# Autodesk Inventor assembly: asmTemp
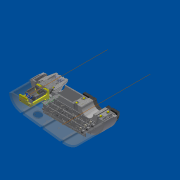
[picture p0: Inventor's stored thumbnail of the model, 180x180]
Saved by Autodesk Inventor 2018 (Build 220112000, 112)
## iProperties
Created: 2019-11-13
Part Number: asmTemp
Document SubType Name: Assembly
Designer: Bunny320
Author: Bunny320
## Documents named in this file (22)
- C:\Users\Bunny320\Desktop\sechs\4-CAD\10-J1.iam
- C:\Users\Bunny320\Desktop\sechs\4-CAD\generated\J1_belt.iam
- C:\Users\Bunny320\Desktop\sechs\4-CAD\standardParts\61814-2RS1\61814-2RS1.iam
- C:\Users\Bunny320\Desktop\sechs\4-CAD\AS5047.ipt
- C:\Users\Bunny320\Desktop\sechs\4-CAD\standardParts\SUNNYSKY-X6215S-kv170\X6215S.ipt
- C:\Users\Bunny320\Desktop\sechs\4-CAD\104-motor-case-new.ipt
- C:\Users\Bunny320\Desktop\sechs\4-CAD\102-top-motor-adapt-big-motor.ipt
- C:\Users\Bunny320\Desktop\sechs\4-CAD\105-flange adapter.ipt
- C:\Users\Bunny320\Documents\Inventor\Content Center Files\R2018\en-US\ISO 10642(2)\ISO 10642  - M3  x  20.ipt
- C:\Users\Bunny320\Documents\Inventor\Content Center Files\R2018\en-US\ISO 4762(1)\DIN EN ISO 4762 - M2 x 6.ipt
- C:\Users\Bunny320\Documents\Inventor\Content Center Files\R2018\en-US\DIN EN ISO 4032\DIN EN ISO 4032 - M2.ipt
- C:\Users\Bunny320\Documents\Inventor\Content Center Files\R2018\en-US\ISO 10642(2)\ISO 10642  - M4  x  16.ipt
- C:\Users\Bunny320\Documents\Inventor\Content Center Files\R2018\en-US\ISO 4762(1)\DIN EN ISO 4762 - M3 x 10.ipt
- C:\Users\Bunny320\Desktop\sechs\4-CAD\standardParts\Pololu mounting hub\pololu-universal-aluminum-mounting-hub-for-6mm-shaft-m3-holes.ipt
- C:\Users\Bunny320\Desktop\sechs\4-CAD\standardParts\61807-2RS1\61807-2RS1.iam
- C:\Users\Bunny320\Desktop\sechs\4-CAD\generated\J1_belt\Design Accelerator\Synchronous Pulley11.ipt
- C:\Users\Bunny320\Desktop\sechs\4-CAD\standardParts\Odrive\PCBasembly_simp.ipt
- C:\Users\Bunny320\Desktop\sechs\4-CAD\motor unit 2820 (J1).iam
- C:\Users\Bunny320\Desktop\sechs\4-CAD\106-pulley adapter.ipt
- C:\Users\Bunny320\Desktop\sechs\4-CAD\112-base middle.ipt
- C:\Users\Bunny320\Desktop\sechs\4-CAD\113-base bottom.ipt
- C:\Users\Bunny320\Desktop\sechs\4-CAD\114-base top.ipt
## Components (47 placed, 21 different names)
1. 112-base middle:1 — Mate:5, Mate:28, Mate:102, Mate:107, Mate:108, Mate:109, Mate:111, Mate:112, Mate:113
2. J1_belt:1 [sub-assembly] — Mate:1, Mate:2, Mate:3, Mate:6, Mate:7, Mate:8, Mate:20, Mate:26, Mate:27, Mate:30, Mate:32, Mate:33, Mate:34, Mate:35, Mate:101, Mate:105, Mate:106
3. 61814-2RS1:1 [sub-assembly] — Mate:2, Mate:8, Mate:110
4. 61814-2RS1:2 [sub-assembly] — Mate:3, Mate:5, Mate:7
5. AS5047:1 — Mate:21, Mate:22, Mate:23, Mate:37, Mate:39, Mate:41, Mate:43
6. X6215S:1 — Mate:24, Mate:25, Mate:26
7. 104-motor-case-new:1 — Mate:20, Mate:21, Mate:22, Mate:23, Mate:24, Mate:25, Mate:36, Mate:38, Mate:40, Mate:42, Mate:45, Mate:47, Mate:49, Mate:51, Mate:52
8. 102-top-motor-adapt-big-motor:1 — Mate:27, Mate:28, Mate:29, Mate:53, Mate:54, Mate:55, Mate:56, Mate:57, Mate:58, Mate:59, Mate:60, Mate:61, Mate:62, Mate:63, Mate:64, Mate:66, Mate:68, Mate:70, Mate:72, Mate:74, Mate:76, Mate:78
9. 105-flange adapter:1 — Mate:30, Mate:105, Mate:106
10. DIN EN ISO 10642 M3  x  20:1 — Mate:32
11. DIN EN ISO 10642 M3  x  20:2 — Mate:33
12. DIN EN ISO 10642 M3  x  20:3 — Mate:34
13. DIN EN ISO 10642 M3  x  20:4 — Mate:35
14. DIN EN ISO 4762 M2 x 6:1 — Mate:36, Mate:37, Mate:50
15. DIN EN ISO 4762 M2 x 6:2 — Mate:38, Mate:39, Mate:46
16. DIN EN ISO 4762 M2 x 6:3 — Mate:40, Mate:41, Mate:44
17. DIN EN ISO 4762 M2 x 6:4 — Mate:42, Mate:43, Mate:48
18. DIN EN ISO 4032 M2:1 — Mate:44, Mate:45
19. DIN EN ISO 4032 M2:2 — Mate:46, Mate:47
20. DIN EN ISO 4032 M2:3 — Mate:48, Mate:49
21. DIN EN ISO 4032 M2:4 — Mate:50, Mate:51
22. DIN EN ISO 4762 M3 x 10:1 — Mate:53, Mate:54
23. DIN EN ISO 4762 M3 x 10:2 — Mate:55, Mate:56
24. DIN EN ISO 4762 M3 x 10:3 — Mate:57, Mate:58
25. DIN EN ISO 4762 M3 x 10:4 — Mate:59, Mate:60
26. DIN EN ISO 4762 M3 x 10:5 — Mate:61, Mate:62
27. DIN EN ISO 4762 M3 x 10:6 — Mate:63, Mate:64
28. DIN EN ISO 4762 M3 x 10:7 — Mate:66
29. DIN EN ISO 4762 M3 x 10:8 — Mate:68
30. DIN EN ISO 4762 M3 x 10:9 — Mate:70
31. DIN EN ISO 4762 M3 x 10:10 — Mate:72
32. DIN EN ISO 4762 M3 x 10:11 — Mate:74
33. DIN EN ISO 4762 M3 x 10:12 — Mate:76
34. DIN EN ISO 4762 M3 x 10:13 — Mate:78
35. motor unit 2820 (J1):1 [sub-assembly] — Flush:4, Mate:92, Mate:100, Mate:101, Mate:102
36. pololu-universal-aluminum-mounting-hub-for-6mm-shaft-m3-holes:1 — Flush:4, Mate:92, Mate:97
37. 61807-2RS1:1 [sub-assembly] — Mate:98, Mate:99, Mate:100, Mate:103, Mate:104
38. Synchronous Pulley1:1 — Mate:97, Mate:98, Mate:99
39. PCBasembly_simp:1 — Mate:112, Mate:113
40. 106-pulley adapter:1 — Mate:103, Mate:104
41. 113-base bottom:1 — Mate:107, Mate:108, Mate:109
42. 114-base top:1 — Mate:110, Mate:111
43. PCBasembly_simp:2
44. PCBasembly_simp:3
45. DIN EN ISO 10642 M4  x  16:1 — Mate:52
46. DIN EN ISO 10642 M4  x  16:2
47. DIN EN ISO 10642 M4  x  16:3
## Component patterns: (4 elements, first: DIN EN ISO 10642 M4  x  16:1)
## Relationships (80: Mate 76, Flush 4)
- [Flush]: 112-base middle:1
- [Flush]: 112-base middle:1
- [Flush]: 112-base middle:1
- Mate:1: J1_belt:1
- Mate:2: J1_belt:1 ↔ 61814-2RS1:1
- Mate:3: J1_belt:1 ↔ 61814-2RS1:2
- Mate:5: 112-base middle:1 ↔ 61814-2RS1:2
- Mate:6: J1_belt:1
- Mate:7: J1_belt:1 ↔ 61814-2RS1:2
- Mate:8: J1_belt:1 ↔ 61814-2RS1:1
- Mate:20: J1_belt:1 ↔ 104-motor-case-new:1
- Mate:21: AS5047:1 ↔ 104-motor-case-new:1
- Mate:22: AS5047:1 ↔ 104-motor-case-new:1
- Mate:23: AS5047:1 ↔ 104-motor-case-new:1
- Mate:24: X6215S:1 ↔ 104-motor-case-new:1
- Mate:25: X6215S:1 ↔ 104-motor-case-new:1
- Mate:26: J1_belt:1 ↔ X6215S:1
- Mate:27: J1_belt:1 ↔ 102-top-motor-adapt-big-motor:1
- Mate:28: 112-base middle:1 ↔ 102-top-motor-adapt-big-motor:1
- Mate:29: 102-top-motor-adapt-big-motor:1
- Mate:30: J1_belt:1 ↔ 105-flange adapter:1
- Mate:32: J1_belt:1 ↔ DIN EN ISO 10642 M3  x  20:1
- Mate:33: J1_belt:1 ↔ DIN EN ISO 10642 M3  x  20:2
- Mate:34: J1_belt:1 ↔ DIN EN ISO 10642 M3  x  20:3
- Mate:35: J1_belt:1 ↔ DIN EN ISO 10642 M3  x  20:4
- Mate:36: 104-motor-case-new:1 ↔ DIN EN ISO 4762 M2 x 6:1
- Mate:37: AS5047:1 ↔ DIN EN ISO 4762 M2 x 6:1
- Mate:38: 104-motor-case-new:1 ↔ DIN EN ISO 4762 M2 x 6:2
- Mate:39: AS5047:1 ↔ DIN EN ISO 4762 M2 x 6:2
- Mate:40: 104-motor-case-new:1 ↔ DIN EN ISO 4762 M2 x 6:3
- Mate:41: AS5047:1 ↔ DIN EN ISO 4762 M2 x 6:3
- Mate:42: 104-motor-case-new:1 ↔ DIN EN ISO 4762 M2 x 6:4
- Mate:43: AS5047:1 ↔ DIN EN ISO 4762 M2 x 6:4
- Mate:44: DIN EN ISO 4762 M2 x 6:3 ↔ DIN EN ISO 4032 M2:1
- Mate:45: 104-motor-case-new:1 ↔ DIN EN ISO 4032 M2:1
- Mate:46: DIN EN ISO 4762 M2 x 6:2 ↔ DIN EN ISO 4032 M2:2
- Mate:47: 104-motor-case-new:1 ↔ DIN EN ISO 4032 M2:2
- Mate:48: DIN EN ISO 4762 M2 x 6:4 ↔ DIN EN ISO 4032 M2:3
- Mate:49: 104-motor-case-new:1 ↔ DIN EN ISO 4032 M2:3
- Mate:50: DIN EN ISO 4762 M2 x 6:1 ↔ DIN EN ISO 4032 M2:4
- Mate:51: 104-motor-case-new:1 ↔ DIN EN ISO 4032 M2:4
- Mate:52: 104-motor-case-new:1 ↔ DIN EN ISO 10642 M4  x  16:1
- Mate:53: 102-top-motor-adapt-big-motor:1 ↔ DIN EN ISO 4762 M3 x 10:1
- Mate:54: 102-top-motor-adapt-big-motor:1 ↔ DIN EN ISO 4762 M3 x 10:1
- Mate:55: 102-top-motor-adapt-big-motor:1 ↔ DIN EN ISO 4762 M3 x 10:2
- Mate:56: 102-top-motor-adapt-big-motor:1 ↔ DIN EN ISO 4762 M3 x 10:2
- Mate:57: 102-top-motor-adapt-big-motor:1 ↔ DIN EN ISO 4762 M3 x 10:3
- Mate:58: 102-top-motor-adapt-big-motor:1 ↔ DIN EN ISO 4762 M3 x 10:3
- Mate:59: 102-top-motor-adapt-big-motor:1 ↔ DIN EN ISO 4762 M3 x 10:4
- Mate:60: 102-top-motor-adapt-big-motor:1 ↔ DIN EN ISO 4762 M3 x 10:4
- Mate:61: 102-top-motor-adapt-big-motor:1 ↔ DIN EN ISO 4762 M3 x 10:5
- Mate:62: 102-top-motor-adapt-big-motor:1 ↔ DIN EN ISO 4762 M3 x 10:5
- Mate:63: 102-top-motor-adapt-big-motor:1 ↔ DIN EN ISO 4762 M3 x 10:6
- Mate:64: 102-top-motor-adapt-big-motor:1 ↔ DIN EN ISO 4762 M3 x 10:6
- Mate:66: 102-top-motor-adapt-big-motor:1 ↔ DIN EN ISO 4762 M3 x 10:7
- Mate:68: 102-top-motor-adapt-big-motor:1 ↔ DIN EN ISO 4762 M3 x 10:8
- Mate:70: 102-top-motor-adapt-big-motor:1 ↔ DIN EN ISO 4762 M3 x 10:9
- Mate:72: 102-top-motor-adapt-big-motor:1 ↔ DIN EN ISO 4762 M3 x 10:10
- Mate:74: 102-top-motor-adapt-big-motor:1 ↔ DIN EN ISO 4762 M3 x 10:11
- Mate:76: 102-top-motor-adapt-big-motor:1 ↔ DIN EN ISO 4762 M3 x 10:12
- Mate:78: 102-top-motor-adapt-big-motor:1 ↔ DIN EN ISO 4762 M3 x 10:13
- Flush:4: motor unit 2820 (J1):1 ↔ pololu-universal-aluminum-mounting-hub-for-6mm-shaft-m3-holes:1
- Mate:92: motor unit 2820 (J1):1 ↔ pololu-universal-aluminum-mounting-hub-for-6mm-shaft-m3-holes:1
- Mate:97: pololu-universal-aluminum-mounting-hub-for-6mm-shaft-m3-holes:1 ↔ Synchronous Pulley1:1
- Mate:98: 61807-2RS1:1 ↔ Synchronous Pulley1:1
- Mate:99: 61807-2RS1:1 ↔ Synchronous Pulley1:1
- Mate:100: motor unit 2820 (J1):1 ↔ 61807-2RS1:1
- Mate:101: J1_belt:1 ↔ motor unit 2820 (J1):1
- Mate:102: 112-base middle:1 ↔ motor unit 2820 (J1):1
- Mate:103: 61807-2RS1:1 ↔ 106-pulley adapter:1
- Mate:104: 61807-2RS1:1 ↔ 106-pulley adapter:1
- Mate:105: J1_belt:1 ↔ 105-flange adapter:1
- Mate:106: J1_belt:1 ↔ 105-flange adapter:1
- Mate:107: 112-base middle:1 ↔ 113-base bottom:1
- Mate:108: 112-base middle:1 ↔ 113-base bottom:1
- Mate:109: 112-base middle:1 ↔ 113-base bottom:1
- Mate:110: 61814-2RS1:1 ↔ 114-base top:1
- Mate:111: 112-base middle:1 ↔ 114-base top:1
- Mate:112: 112-base middle:1 ↔ PCBasembly_simp:1
- Mate:113: 112-base middle:1 ↔ PCBasembly_simp:1
